# Autodesk Inventor assembly: dtmotorgears_MIR1
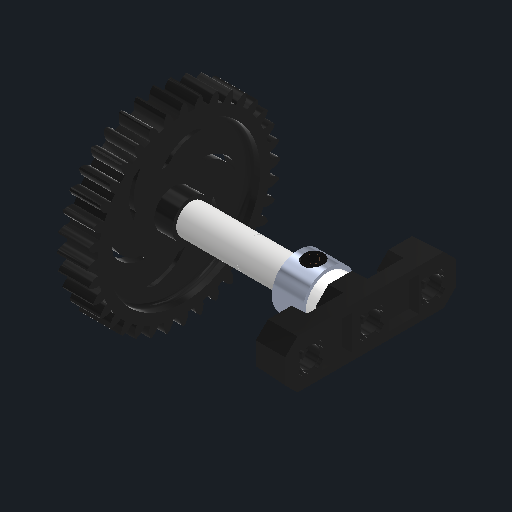
[picture p0: Inventor's stored thumbnail of the model, 512x512]
Saved by Autodesk Inventor 2026.1 (Build 301233000, 233)
## iProperties
Created: 2025-08-03
Part Number: dtmotorgears_MIR1
Document SubType Name: Assembly
Designer: roejo
Author: roejo
## Documents named in this file (9)
- C:\Users\roejo\OneDrive\Documents\2026WorldChampionRobot\Robots\Worlds\Subassemblies\dtmotorgears_MIR1.iam
- C:\Users\roejo\OneDrive\Documents\2026WorldChampionRobot\Library\VEX-CAD-Inventor-1.4.2\Motion\Gears\LS 36T Gear_MIR1.ipt
- C:\Users\roejo\OneDrive\Documents\2026WorldChampionRobot\Library\VEX-CAD-Inventor-1.4.2\Motion\Spacers\Washer Teflon\TWasher .375 OD x .06250.ipt
- C:\Users\roejo\OneDrive\Documents\2026WorldChampionRobot\Library\VEX-CAD-Inventor-1.4.2\Motion\Spacers\Washer Teflon.ipt
- C:\Users\roejo\OneDrive\Documents\2026WorldChampionRobot\Library\VEX-CAD-Inventor-1.4.2\Motion\Spacers\Washer Teflon\TWasher .375 OD x .03125.ipt
- C:\Users\roejo\OneDrive\Documents\2026WorldChampionRobot\Library\VEX-CAD-Inventor-1.4.2\Motion\Shaft LS\Bearing Flat_MIR2.ipt
- C:\Users\roejo\OneDrive\Documents\2026WorldChampionRobot\Library\VEX-CAD-Inventor-1.4.2\Motion\Shaft LS\Shaft Collar Metal\Shaft Collar Set Screw_MIR3.ipt
- C:\Users\roejo\OneDrive\Documents\2026WorldChampionRobot\Library\VEX-CAD-Inventor-1.4.2\Motion\Spacers\thinspacer0.375_MIR1.ipt
- C:\Users\roejo\OneDrive\Documents\2026WorldChampionRobot\Library\VEX-CAD-Inventor-1.4.2\Motion\Spacers\thinspacer0.5_MIR1.ipt
## Components (8 placed, 7 different names)
1. LS 36T Gear_MIR1:1 — Insert:1, Insert:17
2. TWasher .375 OD x .06250:1 — Insert:1
3. TWasher .375 OD x .06250:2 — Insert:11, Insert:10
4. TWasher .375 OD x .03125:3 — Insert:11, Insert:12
5. Bearing Flat_MIR2:1 — Insert:10
6. Shaft Collar Set Screw_MIR3:1 — Insert:12, Insert:15
7. thinspacer0.375_MIR1:1 — Insert:15, Insert:16
8. thinspacer0.5_MIR1:1 — Insert:17, Insert:16
## Relationships (7: Insert 7)
- Insert:1: LS 36T Gear_MIR1:1 ↔ TWasher .375 OD x .06250:1
- Insert:11: TWasher .375 OD x .06250:2 ↔ TWasher .375 OD x .03125:3
- Insert:10: TWasher .375 OD x .06250:2 ↔ Bearing Flat_MIR2:1
- Insert:12: TWasher .375 OD x .03125:3 ↔ Shaft Collar Set Screw_MIR3:1
- Insert:15: Shaft Collar Set Screw_MIR3:1 ↔ thinspacer0.375_MIR1:1
- Insert:17: LS 36T Gear_MIR1:1 ↔ thinspacer0.5_MIR1:1
- Insert:16: thinspacer0.375_MIR1:1 ↔ thinspacer0.5_MIR1:1
